# Autodesk Inventor assembly: 300 mm core xy
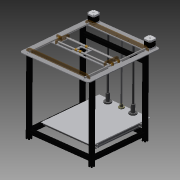
[picture p0: Inventor's stored thumbnail of the model, 180x180]
Saved by Autodesk Inventor 2014 SP1 (Build 180222100, 222)
## iProperties
Created: 2014-09-28
Part Number: 300 mm core xy
Document SubType Name: Assembly
Designer: Mon
Author: Mon
## Documents named in this file (23)
- H:\core xy\300 mm core xy.iam
- H:\core xy\300 mm top plate.ipt
- H:\core xy\2020 extrusion big machine leg.ipt
- H:\core xy\2020 extrusion Y cross big machine.ipt
- H:\core xy\2020 extrusion X cross big machine.ipt
- H:\core xy\300 mm build volume.ipt
- H:\core xy\M1173041- NEMA 17.ipt
- H:\core xy\TR8x1.25 x 450 mm.ipt
- H:\core xy\prototype build plate small.ipt
- H:\core xy\LHFRD10.ipt
- H:\core xy\PSFG10_400.ipt
- H:\core xy\300 mm core xy gantry.ipt
- H:\core xy\300 mm core xy mount.ipt
- H:\core xy\z motor mount.ipt
- H:\core xy\z smooth rod mount.ipt
- H:\core xy\acrylic Y bracket.ipt
- H:\core xy\y rod.ipt
- H:\core xy\x and y bushing.ipt
- H:\core xy\acrylic x bushing bracket.ipt
- H:\core xy\x rod.ipt
- H:\core xy\acrylic X bracket.ipt
- H:\core xy\MTSFR8.ipt
- H:\core xy\print bed frame.iam
## Components (44 placed, 22 different names)
1. 300 mm top plate:1 — Mate:1, Flush:1, Mate:2, Flush:2, Mate:3, Flush:3, Mate:4, Flush:4, Mate:13, Mate:14
2. 2020 extrusion Y cross big machine:2 — Mate:5, Flush:5
3. 2020 extrusion big machine leg:1 — Mate:3, Flush:3, Mate:5, Flush:5, Mate:6, Flush:6
4. 2020 extrusion big machine leg:2 — Mate:1, Flush:1
5. 2020 extrusion big machine leg:3 — Mate:4, Flush:4, Flush:9
6. 2020 extrusion big machine leg:4 — Mate:2, Flush:2, Mate:7, Flush:7, Flush:8
7. 2020 extrusion X cross big machine:1 — Mate:6, Flush:6
8. 2020 extrusion X cross big machine:2 — Mate:7, Flush:7, Mate:8
9. 2020 extrusion Y cross big machine:3 — Mate:8, Flush:8
10. 300 mm build volume:1
11. M1173041- NEMA 17:1 — Mate:11, Mate:12
12. TR8x1.25 x 450 mm:1 — Mate:12
13. LHFRD10:1
14. LHFRD10:2
15. PSFG10_400:1
16. PSFG10_400:2
17. 300 mm core xy gantry:1
18. 300 mm core xy mount:1
19. z motor mount:1 — Mate:11
20. prototype build plate small:1
21. M1173041- NEMA 17:2 — Mate:14
22. M1173041- NEMA 17:3 — Mate:13
23. z smooth rod mount:1
24. z smooth rod mount:2
25. acrylic Y bracket:1
26. acrylic Y bracket:2
27. y rod:1
28. y rod:2
29. x and y bushing:1
30. x and y bushing:2
31. x and y bushing:3
32. acrylic x bushing bracket:1
33. acrylic x bushing bracket:2
34. acrylic x bushing bracket:3
35. x rod:1
36. x rod:2
37. acrylic X bracket:1
38. acrylic X bracket:2
39. x and y bushing:4
40. x and y bushing:5
41. x and y bushing:6
42. 2020 extrusion X cross big machine:3 — Flush:9
43. MTSFR8:1
44. print bed frame:1 [sub-assembly]
## Relationships (21: Mate 12, Flush 9)
- Mate:1: 300 mm top plate:1 ↔ 2020 extrusion big machine leg:2
- Flush:1: 300 mm top plate:1 ↔ 2020 extrusion big machine leg:2
- Mate:2: 300 mm top plate:1 ↔ 2020 extrusion big machine leg:4
- Flush:2: 300 mm top plate:1 ↔ 2020 extrusion big machine leg:4
- Mate:3: 300 mm top plate:1 ↔ 2020 extrusion big machine leg:1
- Flush:3: 300 mm top plate:1 ↔ 2020 extrusion big machine leg:1
- Mate:4: 300 mm top plate:1 ↔ 2020 extrusion big machine leg:3
- Flush:4: 300 mm top plate:1 ↔ 2020 extrusion big machine leg:3
- Mate:5: 2020 extrusion Y cross big machine:2 ↔ 2020 extrusion big machine leg:1
- Flush:5: 2020 extrusion Y cross big machine:2 ↔ 2020 extrusion big machine leg:1
- Mate:6: 2020 extrusion big machine leg:1 ↔ 2020 extrusion X cross big machine:1
- Flush:6: 2020 extrusion big machine leg:1 ↔ 2020 extrusion X cross big machine:1
- Mate:7: 2020 extrusion big machine leg:4 ↔ 2020 extrusion X cross big machine:2
- Flush:7: 2020 extrusion big machine leg:4 ↔ 2020 extrusion X cross big machine:2
- Mate:8: 2020 extrusion X cross big machine:2 ↔ 2020 extrusion Y cross big machine:3
- Flush:8: 2020 extrusion big machine leg:4 ↔ 2020 extrusion Y cross big machine:3
- Mate:11: M1173041- NEMA 17:1 ↔ z motor mount:1
- Mate:12: M1173041- NEMA 17:1 ↔ TR8x1.25 x 450 mm:1
- Mate:13: 300 mm top plate:1 ↔ M1173041- NEMA 17:3
- Mate:14: 300 mm top plate:1 ↔ M1173041- NEMA 17:2
- Flush:9: 2020 extrusion big machine leg:3 ↔ 2020 extrusion X cross big machine:3
